# Autodesk Inventor assembly: pro_complex_frame_assembly
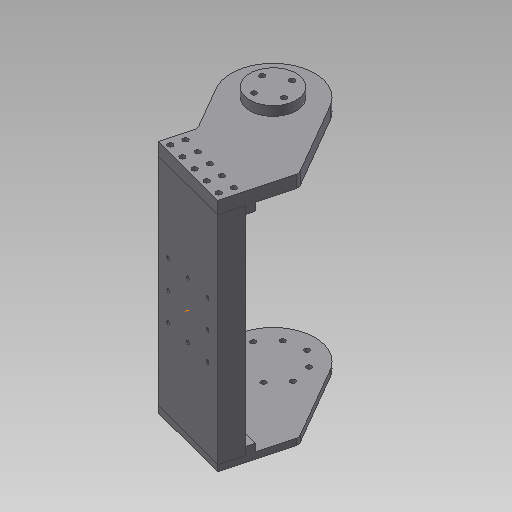
[picture p0: Inventor's stored thumbnail of the model, 512x512]
Saved by Autodesk Inventor 2017 (Build 210142000, 142)
## iProperties
Part Number: pro_complex_frame_assembly
Material: Generisch
Document SubType Name: Assembly
Designer: Max
Mass: 229.195 g
Surface Area: 528.074 cm^2
Volume: 85.8058 cm^3
Density: 2.67109 g/cm^3
Author: Max
## Documents named in this file (5)
- C:\Users\Max\Desktop\SENAI\robot_arm_new\complex_frame\pro_complex_frame_assembly.iam
- C:\Users\Max\Desktop\SENAI\robot_arm_new\complex_frame\pro_complex_frame_part1.ipt
- C:\Users\Max\Desktop\SENAI\robot_arm_new\complex_frame\pro_complex_frame_part2.ipt
- C:\Users\Max\Desktop\SENAI\robot_arm_new\complex_frame\pro_complex_frame_part3.ipt
- C:\Users\Max\Desktop\SENAI\robot_arm_new\dynamixel_pro_frame_shaft.ipt
## Components (4 placed, 4 different names)
1. pro_complex_frame_part1:1 — Passend:1, Passend:2, Passend:3, Passend:4, Passend:5, Passend:6
2. pro_complex_frame_part2:1 — Passend:1, Passend:2, Passend:3, Passend:7, Passend:8, Passend:9
3. pro_complex_frame_part3:1 — Passend:4, Passend:5, Passend:6
4. dynamixel_pro_frame_shaft:1 — Passend:8, Passend:9
## Relationships (9: Mate 9)
- Passend:1 [Mate]: pro_complex_frame_part1:1 ↔ pro_complex_frame_part2:1
- Passend:2 [Mate]: pro_complex_frame_part1:1 ↔ pro_complex_frame_part2:1
- Passend:3 [Mate]: pro_complex_frame_part1:1 ↔ pro_complex_frame_part2:1
- Passend:4 [Mate]: pro_complex_frame_part1:1 ↔ pro_complex_frame_part3:1
- Passend:5 [Mate]: pro_complex_frame_part1:1 ↔ pro_complex_frame_part3:1
- Passend:6 [Mate]: pro_complex_frame_part1:1 ↔ pro_complex_frame_part3:1
- Passend:7 [Mate]: pro_complex_frame_part2:1
- Passend:8 [Mate]: pro_complex_frame_part2:1 ↔ dynamixel_pro_frame_shaft:1
- Passend:9 [Mate]: pro_complex_frame_part2:1 ↔ dynamixel_pro_frame_shaft:1
